# Autodesk Inventor assembly: ShortSupportPlateAssembly
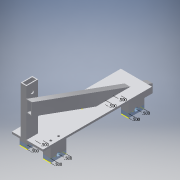
[picture p0: Inventor's stored thumbnail of the model, 180x180]
Saved by Autodesk Inventor 2016 SP1 (Build 200210100, 210)
## iProperties
Created: 2016-02-05
Part Number: ShortSupportPlateAssembly
Document SubType Name: Assembly
Designer: steele
Author: steele
## Documents named in this file (3)
- C:\snobotics\CAD-Development\robSteele\SnoBotics2016\2016-01-31-Lift\ShortSupportPlateAssembly.iam
- C:\snobotics\CAD-Development\robSteele\SnoBotics2016\2016-01-31-Lift\shortSupportPlate.ipt
- C:\snobotics\CAD-Development\robSteele\SnoBotics2016\2015-02-05-RhinoRobotNarrowView\capForLift.ipt
## Components (5 placed, 2 different names)
1. shortSupportPlate:1 — Mate:1, Flush:1, Mate:2, Flush:2, Mate:3, Flush:3, Flush:4, Mate:4, Flush:5, Flush:6, Flush:7, Flush:8, Flush:9, Flush:10
2. capForLift:1 — Mate:1, Flush:1, Flush:8
3. capForLift:2 — Mate:2, Flush:2, Flush:7
4. capForLift:3 — Mate:3, Flush:3, Flush:4, Flush:9
5. capForLift:4 — Mate:4, Flush:5, Flush:6, Flush:10
## Relationships (14: Flush 10, Mate 4)
- Mate:1: shortSupportPlate:1 ↔ capForLift:1
- Flush:1: shortSupportPlate:1 ↔ capForLift:1
- Mate:2: shortSupportPlate:1 ↔ capForLift:2
- Flush:2: shortSupportPlate:1 ↔ capForLift:2
- Mate:3: shortSupportPlate:1 ↔ capForLift:3
- Flush:3: shortSupportPlate:1 ↔ capForLift:3
- Flush:4: shortSupportPlate:1 ↔ capForLift:3
- Mate:4: shortSupportPlate:1 ↔ capForLift:4
- Flush:5: shortSupportPlate:1 ↔ capForLift:4
- Flush:6: shortSupportPlate:1 ↔ capForLift:4
- Flush:7: shortSupportPlate:1 ↔ capForLift:2
- Flush:8: shortSupportPlate:1 ↔ capForLift:1
- Flush:9: shortSupportPlate:1 ↔ capForLift:3
- Flush:10: shortSupportPlate:1 ↔ capForLift:4
